# Autodesk Inventor assembly: Segment_2
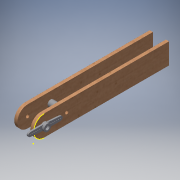
[picture p0: Inventor's stored thumbnail of the model, 180x180]
Saved by Autodesk Inventor 2017 (Build 210142000, 142)
## iProperties
Part Number: Segment_2
Material: Ogólny
Document SubType Name: Assembly
Designer: Damian
Author: Damian
## Documents named in this file (5)
- C:\Users\Damian\Documents\Inventor\Nowe\2.0\Segment_2.iam
- C:\Users\Damian\Documents\Inventor\Nowe\2.0\Część3.ipt
- C:\Users\Damian\Documents\Inventor\Nowe\2.0\Część4.ipt
- C:\Users\Damian\Documents\Inventor\Nowe\2.0\tuleja12,5.ipt
- C:\Users\Damian\Documents\Inventor\Nowe\2.0\Micro Servo 9g Arm.ipt
## Components (4 placed, 4 different names)
1. Część3:1 — Sztywne:1, Sztywne:3
2. Część4:1 — Sztywne:1, Sztywne:2
3. tuleja12,5:1 — Sztywne:2
4. Micro Servo 9g Arm:1 — Sztywne:3
## Relationships (3: WeldJoint 3)
- Sztywne:1 [WeldJoint] (12.5 mm): Część3:1 ↔ Część4:1
- Sztywne:2 [WeldJoint]: Część4:1 ↔ tuleja12,5:1
- Sztywne:3 [WeldJoint]: Część3:1 ↔ Micro Servo 9g Arm:1
